# Autodesk Inventor assembly: Acetal_Washer_16
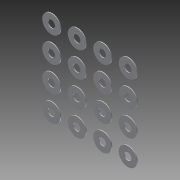
[picture p0: Inventor's stored thumbnail of the model, 180x180]
Saved by Autodesk Inventor 2013 (Build 170138000, 138)
## iProperties
Created: 2014-04-28
Part Number: Acetal_Washer_16
Document SubType Name: Assembly
Designer: andou
Author: andou
## Documents named in this file (2)
- C:\Users\andou\Documents\GitHub\Robotics-Project\design\RoboticsProject\project_4\cnc_data\Acetal_Washer_16.iam
- C:\Users\andou\Documents\GitHub\Robotics-Project\design\RoboticsProject\project_4\cnc_data\Leg_Acetal_Washer.ipt
## Components (16 placed, 1 different names)
1. Leg_Acetal_Washer:1
2. Leg_Acetal_Washer:2
3. Leg_Acetal_Washer:3
4. Leg_Acetal_Washer:4
5. Leg_Acetal_Washer:5
6. Leg_Acetal_Washer:6
7. Leg_Acetal_Washer:7
8. Leg_Acetal_Washer:8
9. Leg_Acetal_Washer:9
10. Leg_Acetal_Washer:10
11. Leg_Acetal_Washer:11
12. Leg_Acetal_Washer:12
13. Leg_Acetal_Washer:13
14. Leg_Acetal_Washer:14
15. Leg_Acetal_Washer:15
16. Leg_Acetal_Washer:16
## Component patterns: (16 elements, first: Leg_Acetal_Washer:1)
